# Autodesk Inventor assembly: motorizedSwitchHanger
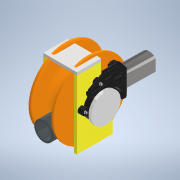
[picture p0: Inventor's stored thumbnail of the model, 180x180]
Saved by Autodesk Inventor 2020.2 (Build 242310000, 310)
## iProperties
Created: 2020-01-06
Part Number: motorizedSwitchHanger
Document SubType Name: Assembly
Designer: steele
Author: steele
## Documents named in this file (10)
- C:\git\CAD-Development\robSteele\2020 Lift Mechanism\motorizedSwitchHanger.iam
- C:\git\CAD-Development\robSteele\2020 Lift Mechanism\switchHangingPipe.ipt
- C:\git\CAD-Development\robSteele\2020 Lift Mechanism\wheelForHangingAndMoving.ipt
- C:\git\CAD-Development\robSteele\2020 Lift Mechanism\plateForHangingMechanism.ipt
- C:\git\CAD-Development\robSteele\2020 Lift Mechanism\am-2986 FR8ZZ Hex Bearing.ipt
- C:\git\CAD-Development\robSteele\2020 Lift Mechanism\am-2235a.iam
- C:\git\CAD-Development\robSteele\2020 Lift Mechanism\motorizedSwitchHanger\Design Accelerator\Bolted Connection1.iam
- C:\git\CAD-Development\robSteele\2020 Lift Mechanism\washerAndThrustBearingAssembly.iam
- C:\git\CAD-Development\robSteele\2020 Lift Mechanism\topOfLiftFrame.ipt
- C:\git\CAD-Development\robSteele\2020 Lift Mechanism\hexShaft.ipt
## Components (11 placed, 9 different names)
1. switchHangingPipe:1 — Flush:1, Flush:2, Flush:3
2. wheelForHangingAndMoving:1 — Flush:1, Flush:2, Flush:3, Insert:3, Mate:5, Mate:8, Insert:4
3. plateForHangingMechanism:1 — Insert:1, Insert:3, Mate:5, Flush:4
4. plateForHangingMechanism:2 — Insert:2, Mate:8, Insert:4, Mate:9, Insert:6
5. am-2986 FR8ZZ Hex Bearing:1 — Insert:1, Insert:5
6. am-2235a:1 [sub-assembly] — Insert:2, Mate:10, Mate:11, Flush:5, Flush:6
7. Bolted Connection:1 [sub-assembly] — Mate:9, Mate:10
8. washerAndThrustBearingAssembly:1 [sub-assembly] — Insert:5
9. washerAndThrustBearingAssembly:2 [sub-assembly] — Insert:6
10. topOfLiftFrame:1 — Flush:4
11. hexShaft:1 — Mate:11, Flush:5, Flush:6
## Relationships (17: Flush 6, Insert 6, Mate 5)
- Flush:1: switchHangingPipe:1 ↔ wheelForHangingAndMoving:1
- Flush:2: switchHangingPipe:1 ↔ wheelForHangingAndMoving:1
- Flush:3 (38.1 mm): switchHangingPipe:1 ↔ wheelForHangingAndMoving:1
- Insert:1: plateForHangingMechanism:1 ↔ am-2986 FR8ZZ Hex Bearing:1
- Insert:2 (-6.477 mm): plateForHangingMechanism:2 ↔ am-2235a:1
- Insert:3 (3.81 mm): wheelForHangingAndMoving:1 ↔ plateForHangingMechanism:1
- Mate:5: wheelForHangingAndMoving:1 ↔ plateForHangingMechanism:1
- Mate:8: wheelForHangingAndMoving:1 ↔ plateForHangingMechanism:2
- Insert:4 (3.81 mm): wheelForHangingAndMoving:1 ↔ plateForHangingMechanism:2
- Mate:9: plateForHangingMechanism:2 ↔ Bolted Connection:1
- Mate:10: am-2235a:1 ↔ Bolted Connection:1
- Insert:5: am-2986 FR8ZZ Hex Bearing:1 ↔ washerAndThrustBearingAssembly:1
- Insert:6: plateForHangingMechanism:2 ↔ washerAndThrustBearingAssembly:2
- Flush:4: plateForHangingMechanism:1 ↔ topOfLiftFrame:1
- Mate:11: am-2235a:1 ↔ hexShaft:1
- Flush:5: am-2235a:1 ↔ hexShaft:1
- Flush:6: am-2235a:1 ↔ hexShaft:1
